# Autodesk Inventor assembly: UpperArmActuatorBase
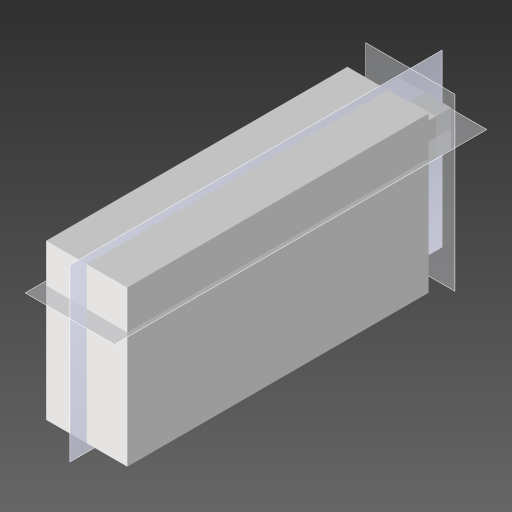
[picture p0: Inventor's stored thumbnail of the model, 512x512]
Saved by Autodesk Inventor 2023 (Build 270158000, 158)
## iProperties
Created: 2023-03-23
Part Number: UpperArmActuatorBase
Document SubType Name: Assembly
Designer: Val
Author: Val
## Documents named in this file (3)
- C:\Users\Val\Desktop\str1ker\description\models\src\UpperArmActuatorBase.iam
- C:\Users\Val\Desktop\str1ker\parts\external\UpperArmActuatorBody.ipt
- C:\Users\Val\Desktop\str1ker\description\models\src\UpperArmActuatorBaseBoundingBox.ipt
## Components (2 placed, 2 different names)
1. UpperArmActuatorBody:1 — Mate:1, Angle:1, Angle:2, Flush:2, Flush:3
2. UpperArmActuatorBaseBoundingBox:1 — Flush:1, Flush:2, Flush:3
## Relationships (6: Flush 3, Angle 2, Mate 1)
- Mate:1: UpperArmActuatorBody:1
- Angle:1 (0 deg): UpperArmActuatorBody:1
- Angle:2 (180 deg): UpperArmActuatorBody:1
- Flush:1: UpperArmActuatorBaseBoundingBox:1
- Flush:2: UpperArmActuatorBody:1 ↔ UpperArmActuatorBaseBoundingBox:1
- Flush:3: UpperArmActuatorBody:1 ↔ UpperArmActuatorBaseBoundingBox:1
